# Autodesk Inventor assembly: Helix DLP
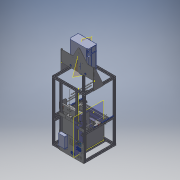
[picture p0: Inventor's stored thumbnail of the model, 180x180]
Saved by Autodesk Inventor 2019 (Build 230136000, 136)
## iProperties
Created: 2020-03-07
Part Number: Helix DLP
Document SubType Name: Assembly
Designer: Vijay
Author: Vijay
## Documents named in this file (32)
- C:\Users\Vijay\Documents\CAD Files\Helix DLP\Helix DLP.iam
- C:\Users\Vijay\Documents\CAD Files\Helix DLP\Helix DLP Z Stage.iam
- C:\Users\Vijay\Documents\CAD Files\Helix DLP\mgn12-linear-guide-subassembly-with-configurable-rail-length-1.snapshot.8\MGN12 LINEAR GUIDE RAIL, CONFIGURABLE, 500 mm.ipt
- C:\Users\Vijay\Documents\CAD Files\Helix DLP\3030-aluminum-extrusion-profile-2.snapshot.4\30X30 - T-slot - Aluminium Profile.ipt
- C:\Users\Vijay\Documents\CAD Files\Helix DLP\3030-aluminum-extrusion-profile-2.snapshot.4\30X30 - T-slot - Aluminium Profile_CPY.ipt
- C:\Users\Vijay\Documents\CAD Files\Helix DLP\3030-aluminum-extrusion-profile-2.snapshot.4\30X30 - T-slot - Aluminium Profile_CPY_CPY.ipt
- C:\Users\Vijay\Documents\CAD Files\Helix DLP\M1173041- NEMA 17 Screw rod.ipt
- C:\Users\Vijay\Documents\CAD Files\Helix DLP\Motor Brace_1.ipt
- C:\Users\Vijay\Documents\CAD Files\Helix DLP\Motor_brace_2.ipt
- C:\Users\Vijay\Documents\CAD Files\Helix DLP\motor_brace_3.ipt
- C:\Users\Vijay\Documents\CAD Files\Helix DLP\Tank2.ipt
- C:\Users\Vijay\Documents\CAD Files\Helix DLP\3030-aluminum-extrusion-profile-2.snapshot.4\30X30 - T-slot - Aluminium Profile_CPY_CPY_CPY.ipt
- C:\Users\Vijay\Documents\CAD Files\Helix DLP\mgn12-linear-guide-subassembly-with-configurable-rail-length-1.snapshot.8\MGN12H, LINEAR GUIDE BLOCK.ipt
- C:\Users\Vijay\Documents\CAD Files\Helix DLP\Wiper_Arm_1.ipt
- C:\Users\Vijay\Documents\CAD Files\Helix DLP\mgn12-linear-guide-subassembly-with-configurable-rail-length-1.snapshot.8\MGN12 LINEAR GUIDE RAIL, CONFIGURABLE, 500 mm_CPY.ipt
- C:\Users\Vijay\Documents\CAD Files\Helix DLP\wiper motor holder.ipt
- C:\Users\Vijay\Documents\CAD Files\Julia Extended Rev19\Julia Chassi(Chamfered)\Julia Chassi(Chamfered)\Julia 3D model\Z Motor Screw.ipt
- C:\Users\Vijay\Documents\CAD Files\Helix DLP\Wiper nut holder.ipt
- C:\Users\Vijay\Documents\CAD Files\Helix DLP\Rain T Slot.ipt
- C:\Users\Vijay\Documents\CAD Files\Helix DLP\Projector.ipt
- C:\Users\Vijay\Documents\CAD Files\Helix DLP\ProjectorMount 1.ipt
- C:\Users\Vijay\Documents\CAD Files\Helix DLP\Projector mount side.ipt
- C:\Users\Vijay\Documents\CAD Files\Helix DLP\SIde Actylic.ipt
- C:\Users\Vijay\Documents\CAD Files\Helix DLP\wiper.ipt
- C:\Users\Vijay\Documents\CAD Files\Helix DLP\wiper 2.ipt
- C:\Users\Vijay\Documents\CAD Files\Helix DLP\Electronics Base.ipt
- C:\Users\Vijay\Documents\CAD Files\Helix DLP\ArduinoUno.ipt
- C:\Users\Vijay\Documents\CAD Files\Helix DLP\V8_AC switch_1.ipt
- C:\Users\Vijay\Documents\CAD Files\Helix DLP\Raspberry Pi 3 Model B+ Reference Model.ipt
- C:\Users\Vijay\Documents\CAD Files\Helix DLP\24v Smps.ipt
- C:\Users\Vijay\Documents\CAD Files\Helix DLP\Limit Switch (1).ipt
- C:\Users\Vijay\Documents\CAD Files\Helix DLP\Z limit switch holder.ipt
## Components (60 placed, 31 different names)
1. Helix DLP Z Stage:1 [sub-assembly] — Mate:1, Mate:2, Mate:3, Mate:19, Angle:1, Mate:34, Mate:35, Angle:4
2. MGN12 LINEAR GUIDE RAIL, CONFIGURABLE, 500 mm:1 — Flush:1, Flush:2, Mate:3, Mate:4, Flush:13
3. MGN12 LINEAR GUIDE RAIL, CONFIGURABLE, 500 mm:2 — Flush:1, Flush:2, Mate:1, Mate:2, Mate:5, Flush:14, Flush:15
4. 30X30 - T-slot - Aluminium Profile:1 — Mate:5, Flush:7, Flush:9, Flush:14, Flush:15, Mate:7, Mate:87, Flush:81, Flush:82
5. 30X30 - T-slot - Aluminium Profile:2 — Mate:4, Flush:8, Flush:13, Mate:6, Flush:17, Flush:39
6. 30X30 - T-slot - Aluminium Profile:3 — Flush:4, Flush:5, Flush:7, Flush:9, Flush:11, Mate:7, Mate:8, Flush:18, Flush:19, Mate:10, Flush:36, Flush:56, Mate:50, Flush:80
7. 30X30 - T-slot - Aluminium Profile:4 — Flush:4, Flush:8, Flush:10, Mate:6, Flush:17, Mate:72
8. 30X30 - T-slot - Aluminium Profile:5 — Flush:5, Flush:6, Flush:10, Flush:12, Flush:20, Flush:21, Flush:25, Flush:37, Mate:17, Mate:22, Flush:44, Mate:43
9. 30X30 - T-slot - Aluminium Profile:6 — Flush:6, Flush:11, Flush:12, Mate:9, Mate:10, Mate:16, Flush:32, Flush:33, Mate:18, Mate:23, Flush:45, Mate:41, Flush:74
10. 30X30 - T-slot - Aluminium Profile_CPY:1 — Mate:8, Flush:18, Flush:19
11. 30X30 - T-slot - Aluminium Profile_CPY:2 — Flush:20, Flush:21, Mate:9, Mate:11, Flush:22, Flush:23, Flush:24, Mate:12
12. 30X30 - T-slot - Aluminium Profile_CPY_CPY:1 — Mate:11, Flush:22, Flush:23
13. 30X30 - T-slot - Aluminium Profile_CPY_CPY:2 — Flush:24, Mate:12, Flush:25, Flush:67
14. 30X30 - T-slot - Aluminium Profile_CPY:3 — Flush:30, Mate:15, Flush:31, Flush:79
15. 30X30 - T-slot - Aluminium Profile_CPY:4 — Flush:29, Mate:16, Flush:32, Mate:37, Flush:53
16. 30X30 - T-slot - Aluminium Profile_CPY_CPY:3 — Flush:31, Flush:33, Mate:38
17. 30X30 - T-slot - Aluminium Profile_CPY_CPY:4 — Flush:29, Flush:30, Mate:15, Mate:39
18. 30X30 - T-slot - Aluminium Profile_CPY_CPY:5 — Flush:37, Mate:17, Flush:38, Flush:55, Mate:42
19. 30X30 - T-slot - Aluminium Profile_CPY_CPY:6 — Flush:36, Mate:18, Flush:38, Mate:40, Flush:54, Mate:47
20. M1173041- NEMA 17 Screw rod:1 — Mate:19, Angle:1, Flush:40
21. Motor Brace_1:1 — Flush:39, Mate:21
22. Motor_brace_2:1 — Flush:40, Flush:41, Mate:20, Flush:42
23. motor_brace_3:1 — Flush:41
24. motor_brace_3:2 — Mate:20, Mate:21, Flush:42
25. Tank2:1 — Mate:24, Mate:33, Mate:34, Mate:35, Angle:3, Mate:68
26. 30X30 - T-slot - Aluminium Profile_CPY_CPY_CPY:1 — Mate:22, Flush:44, Flush:46, Flush:65
27. 30X30 - T-slot - Aluminium Profile_CPY_CPY_CPY:2 — Mate:23, Flush:45, Flush:46, Mate:24
28. MGN12H, LINEAR GUIDE BLOCK:1 — Flush:49, Mate:45, Mate:73
29. MGN12H, LINEAR GUIDE BLOCK:2 — Flush:49, Flush:50, Mate:44, Mate:48, Mate:64, Mate:65
30. Wiper_Arm_1:1 — Flush:50, Mate:33, Mate:51, Mate:52, Flush:59, Flush:61, Mate:64, Mate:65, Flush:77
31. 30X30 - T-slot - Aluminium Profile_CPY_CPY:7 — Flush:51, Mate:38
32. 30X30 - T-slot - Aluminium Profile_CPY_CPY:8 — Flush:51, Mate:37, Flush:53, Mate:39
33. M1173041- NEMA 17 Screw rod:2 — Mate:47, Mate:49, Mate:50, Flush:57, Flush:60, Mate:55
34. MGN12 LINEAR GUIDE RAIL, CONFIGURABLE, 500 mm_CPY:1 — Mate:40, Flush:54, Mate:41, Mate:44, Mate:48
35. MGN12 LINEAR GUIDE RAIL, CONFIGURABLE, 500 mm_CPY:2 — Flush:55, Mate:42, Mate:43, Mate:45, Mate:73
36. wiper motor holder:1 — Flush:56, Mate:49, Flush:57
37. Z Motor Screw:1 — Mate:53, Mate:54, Mate:55, Mate:56
38. motor_brace_3:3 — Mate:52, Flush:58, Flush:59
39. motor_brace_3:4 — Mate:51, Flush:58, Flush:60, Flush:61, Flush:62, Angle:2
40. Wiper nut holder:1 — Flush:62, Mate:53, Mate:54, Mate:56, Angle:2
41. Rain T Slot:1 — Flush:65
42. Projector:1 — Angle:3, Angle:4, Mate:68, Flush:68, Mate:70, Angle:5, Mate:74
43. ProjectorMount 1:1 — Flush:67, Flush:68, Flush:69, Mate:69, Flush:72, Flush:73, Mate:71, Mate:74
44. Projector mount side:1 — Flush:69, Flush:70, Flush:71
45. Projector mount side:2 — Flush:70, Flush:71, Mate:69, Flush:72, Flush:73
46. SIde Actylic:1 — Flush:74, Flush:75, Flush:76
47. SIde Actylic:2 — Mate:72, Flush:75, Flush:76
48. wiper:1 — Flush:77, Flush:78
49. wiper 2:1 — Flush:78
50. Rain T Slot:2
51. Rain T Slot:3
52. Rain T Slot:4
53. Electronics Base:1 — Mate:75, Mate:76, Mate:77, Mate:78, Mate:79, Mate:80, Mate:81, Mate:82, Mate:83, Mate:84, Mate:85, Mate:86, Mate:87, Flush:79, Flush:80
54. ArduinoUno:1 — Mate:76, Mate:77, Mate:85
55. V8_AC switch_1:1 — Mate:81, Mate:82, Mate:84
56. Raspberry Pi 3 Model B+ Reference Model:1 — Mate:78, Mate:79, Mate:86
57. 24v Smps:1 — Mate:75, Mate:80, Mate:83
58. Limit Switch (1):1
59. Limit Switch (1):2
60. Z limit switch holder:1 — Flush:81, Flush:82
## Relationships (144: Flush 71, Mate 68, Angle 5)
- Flush:1: MGN12 LINEAR GUIDE RAIL, CONFIGURABLE, 500 mm:1 ↔ MGN12 LINEAR GUIDE RAIL, CONFIGURABLE, 500 mm:2
- Flush:2: MGN12 LINEAR GUIDE RAIL, CONFIGURABLE, 500 mm:1 ↔ MGN12 LINEAR GUIDE RAIL, CONFIGURABLE, 500 mm:2
- Mate:1: Helix DLP Z Stage:1 ↔ MGN12 LINEAR GUIDE RAIL, CONFIGURABLE, 500 mm:2
- Mate:2: Helix DLP Z Stage:1 ↔ MGN12 LINEAR GUIDE RAIL, CONFIGURABLE, 500 mm:2
- Mate:3: Helix DLP Z Stage:1 ↔ MGN12 LINEAR GUIDE RAIL, CONFIGURABLE, 500 mm:1
- Mate:4: MGN12 LINEAR GUIDE RAIL, CONFIGURABLE, 500 mm:1 ↔ 30X30 - T-slot - Aluminium Profile:2
- Mate:5: MGN12 LINEAR GUIDE RAIL, CONFIGURABLE, 500 mm:2 ↔ 30X30 - T-slot - Aluminium Profile:1
- Flush:4: 30X30 - T-slot - Aluminium Profile:3 ↔ 30X30 - T-slot - Aluminium Profile:4
- Flush:5: 30X30 - T-slot - Aluminium Profile:3 ↔ 30X30 - T-slot - Aluminium Profile:5
- Flush:6: 30X30 - T-slot - Aluminium Profile:5 ↔ 30X30 - T-slot - Aluminium Profile:6
- Flush:7: 30X30 - T-slot - Aluminium Profile:1 ↔ 30X30 - T-slot - Aluminium Profile:3
- Flush:8: 30X30 - T-slot - Aluminium Profile:2 ↔ 30X30 - T-slot - Aluminium Profile:4
- Flush:9: 30X30 - T-slot - Aluminium Profile:1 ↔ 30X30 - T-slot - Aluminium Profile:3
- Flush:10: 30X30 - T-slot - Aluminium Profile:4 ↔ 30X30 - T-slot - Aluminium Profile:5
- Flush:11: 30X30 - T-slot - Aluminium Profile:3 ↔ 30X30 - T-slot - Aluminium Profile:6
- Flush:12: 30X30 - T-slot - Aluminium Profile:5 ↔ 30X30 - T-slot - Aluminium Profile:6
- Flush:13 (9.0175 mm): MGN12 LINEAR GUIDE RAIL, CONFIGURABLE, 500 mm:1 ↔ 30X30 - T-slot - Aluminium Profile:2
- Flush:14 (9.0175 mm): MGN12 LINEAR GUIDE RAIL, CONFIGURABLE, 500 mm:2 ↔ 30X30 - T-slot - Aluminium Profile:1
- Flush:15 (-50 mm): MGN12 LINEAR GUIDE RAIL, CONFIGURABLE, 500 mm:2 ↔ 30X30 - T-slot - Aluminium Profile:1
- Mate:6 (100 mm): 30X30 - T-slot - Aluminium Profile:2 ↔ 30X30 - T-slot - Aluminium Profile:4
- Mate:7 (100 mm): 30X30 - T-slot - Aluminium Profile:1 ↔ 30X30 - T-slot - Aluminium Profile:3
- Flush:17: 30X30 - T-slot - Aluminium Profile:2 ↔ 30X30 - T-slot - Aluminium Profile:4
- Mate:8: 30X30 - T-slot - Aluminium Profile:3 ↔ 30X30 - T-slot - Aluminium Profile_CPY:1
- Flush:18: 30X30 - T-slot - Aluminium Profile:3 ↔ 30X30 - T-slot - Aluminium Profile_CPY:1
- Flush:19: 30X30 - T-slot - Aluminium Profile:3 ↔ 30X30 - T-slot - Aluminium Profile_CPY:1
- Flush:20: 30X30 - T-slot - Aluminium Profile:5 ↔ 30X30 - T-slot - Aluminium Profile_CPY:2
- Flush:21: 30X30 - T-slot - Aluminium Profile:5 ↔ 30X30 - T-slot - Aluminium Profile_CPY:2
- Mate:9: 30X30 - T-slot - Aluminium Profile:6 ↔ 30X30 - T-slot - Aluminium Profile_CPY:2
- Mate:10 (500 mm): 30X30 - T-slot - Aluminium Profile:3 ↔ 30X30 - T-slot - Aluminium Profile:6
- Mate:11: 30X30 - T-slot - Aluminium Profile_CPY:2 ↔ 30X30 - T-slot - Aluminium Profile_CPY_CPY:1
- Flush:22: 30X30 - T-slot - Aluminium Profile_CPY:2 ↔ 30X30 - T-slot - Aluminium Profile_CPY_CPY:1
- Flush:23: 30X30 - T-slot - Aluminium Profile_CPY:2 ↔ 30X30 - T-slot - Aluminium Profile_CPY_CPY:1
- Flush:24: 30X30 - T-slot - Aluminium Profile_CPY:2 ↔ 30X30 - T-slot - Aluminium Profile_CPY_CPY:2
- Mate:12: 30X30 - T-slot - Aluminium Profile_CPY:2 ↔ 30X30 - T-slot - Aluminium Profile_CPY_CPY:2
- Flush:25: 30X30 - T-slot - Aluminium Profile:5 ↔ 30X30 - T-slot - Aluminium Profile_CPY_CPY:2
- [Mate]: 30X30 - T-slot - Aluminium Profile_CPY:4 ↔ 30X30 - T-slot - Aluminium Profile_CPY_CPY:3
- [Flush]: 30X30 - T-slot - Aluminium Profile_CPY:4 ↔ 30X30 - T-slot - Aluminium Profile_CPY_CPY:3
- [Flush]: 30X30 - T-slot - Aluminium Profile_CPY:4 ↔ 30X30 - T-slot - Aluminium Profile_CPY_CPY:3
- [Flush]: 30X30 - T-slot - Aluminium Profile_CPY:4 ↔ 30X30 - T-slot - Aluminium Profile_CPY_CPY:4
- [Mate]: 30X30 - T-slot - Aluminium Profile_CPY:4 ↔ 30X30 - T-slot - Aluminium Profile_CPY_CPY:4
- Flush:29: 30X30 - T-slot - Aluminium Profile_CPY:4 ↔ 30X30 - T-slot - Aluminium Profile_CPY_CPY:4
- Flush:30: 30X30 - T-slot - Aluminium Profile_CPY:3 ↔ 30X30 - T-slot - Aluminium Profile_CPY_CPY:4
- Mate:15: 30X30 - T-slot - Aluminium Profile_CPY:3 ↔ 30X30 - T-slot - Aluminium Profile_CPY_CPY:4
- Mate:16: 30X30 - T-slot - Aluminium Profile:6 ↔ 30X30 - T-slot - Aluminium Profile_CPY:4
- Flush:31: 30X30 - T-slot - Aluminium Profile_CPY:3 ↔ 30X30 - T-slot - Aluminium Profile_CPY_CPY:3
- Flush:32: 30X30 - T-slot - Aluminium Profile:6 ↔ 30X30 - T-slot - Aluminium Profile_CPY:4
- Flush:33: 30X30 - T-slot - Aluminium Profile:6 ↔ 30X30 - T-slot - Aluminium Profile_CPY_CPY:3
- Flush:36: 30X30 - T-slot - Aluminium Profile:3 ↔ 30X30 - T-slot - Aluminium Profile_CPY_CPY:6
- Flush:37: 30X30 - T-slot - Aluminium Profile:5 ↔ 30X30 - T-slot - Aluminium Profile_CPY_CPY:5
- Mate:17: 30X30 - T-slot - Aluminium Profile:5 ↔ 30X30 - T-slot - Aluminium Profile_CPY_CPY:5
- Mate:18: 30X30 - T-slot - Aluminium Profile:6 ↔ 30X30 - T-slot - Aluminium Profile_CPY_CPY:6
- Flush:38: 30X30 - T-slot - Aluminium Profile_CPY_CPY:5 ↔ 30X30 - T-slot - Aluminium Profile_CPY_CPY:6
- Mate:19: Helix DLP Z Stage:1 ↔ M1173041- NEMA 17 Screw rod:1
- Flush:39: 30X30 - T-slot - Aluminium Profile:2 ↔ Motor Brace_1:1
- Angle:1 (0 deg): Helix DLP Z Stage:1 ↔ M1173041- NEMA 17 Screw rod:1
- Flush:40: M1173041- NEMA 17 Screw rod:1 ↔ Motor_brace_2:1
- Flush:41: Motor_brace_2:1 ↔ motor_brace_3:1
- Mate:20: Motor_brace_2:1 ↔ motor_brace_3:2
- Mate:21: Motor Brace_1:1 ↔ motor_brace_3:2
- Flush:42: Motor_brace_2:1 ↔ motor_brace_3:2
- Mate:22: 30X30 - T-slot - Aluminium Profile:5 ↔ 30X30 - T-slot - Aluminium Profile_CPY_CPY_CPY:1
- Flush:44: 30X30 - T-slot - Aluminium Profile:5 ↔ 30X30 - T-slot - Aluminium Profile_CPY_CPY_CPY:1
- Mate:23: 30X30 - T-slot - Aluminium Profile:6 ↔ 30X30 - T-slot - Aluminium Profile_CPY_CPY_CPY:2
- Flush:45: 30X30 - T-slot - Aluminium Profile:6 ↔ 30X30 - T-slot - Aluminium Profile_CPY_CPY_CPY:2
- Flush:46: 30X30 - T-slot - Aluminium Profile_CPY_CPY_CPY:1 ↔ 30X30 - T-slot - Aluminium Profile_CPY_CPY_CPY:2
- Mate:24: Tank2:1 ↔ 30X30 - T-slot - Aluminium Profile_CPY_CPY_CPY:2
- Flush:49: MGN12H, LINEAR GUIDE BLOCK:1 ↔ MGN12H, LINEAR GUIDE BLOCK:2
- Flush:50: MGN12H, LINEAR GUIDE BLOCK:2 ↔ Wiper_Arm_1:1
- Mate:33 (9 mm): Tank2:1 ↔ Wiper_Arm_1:1
- Mate:34 (10 mm): Helix DLP Z Stage:1 ↔ Tank2:1
- Mate:35 (10 mm): Helix DLP Z Stage:1 ↔ Tank2:1
- Flush:51: 30X30 - T-slot - Aluminium Profile_CPY_CPY:7 ↔ 30X30 - T-slot - Aluminium Profile_CPY_CPY:8
- Mate:37: 30X30 - T-slot - Aluminium Profile_CPY:4 ↔ 30X30 - T-slot - Aluminium Profile_CPY_CPY:8
- Flush:53: 30X30 - T-slot - Aluminium Profile_CPY:4 ↔ 30X30 - T-slot - Aluminium Profile_CPY_CPY:8
- Mate:38 (120 mm): 30X30 - T-slot - Aluminium Profile_CPY_CPY:3 ↔ 30X30 - T-slot - Aluminium Profile_CPY_CPY:7
- Mate:39 (120 mm): 30X30 - T-slot - Aluminium Profile_CPY_CPY:4 ↔ 30X30 - T-slot - Aluminium Profile_CPY_CPY:8
- Mate:40: 30X30 - T-slot - Aluminium Profile_CPY_CPY:6 ↔ MGN12 LINEAR GUIDE RAIL, CONFIGURABLE, 500 mm_CPY:1
- Flush:54 (9.018 mm): 30X30 - T-slot - Aluminium Profile_CPY_CPY:6 ↔ MGN12 LINEAR GUIDE RAIL, CONFIGURABLE, 500 mm_CPY:1
- Mate:41: 30X30 - T-slot - Aluminium Profile:6 ↔ MGN12 LINEAR GUIDE RAIL, CONFIGURABLE, 500 mm_CPY:1
- Flush:55 (9.018 mm): 30X30 - T-slot - Aluminium Profile_CPY_CPY:5 ↔ MGN12 LINEAR GUIDE RAIL, CONFIGURABLE, 500 mm_CPY:2
- Mate:42: 30X30 - T-slot - Aluminium Profile_CPY_CPY:5 ↔ MGN12 LINEAR GUIDE RAIL, CONFIGURABLE, 500 mm_CPY:2
- Mate:43: 30X30 - T-slot - Aluminium Profile:5 ↔ MGN12 LINEAR GUIDE RAIL, CONFIGURABLE, 500 mm_CPY:2
- Mate:44: MGN12H, LINEAR GUIDE BLOCK:2 ↔ MGN12 LINEAR GUIDE RAIL, CONFIGURABLE, 500 mm_CPY:1
- Mate:45: MGN12H, LINEAR GUIDE BLOCK:1 ↔ MGN12 LINEAR GUIDE RAIL, CONFIGURABLE, 500 mm_CPY:2
- Flush:56: 30X30 - T-slot - Aluminium Profile:3 ↔ wiper motor holder:1
- Mate:47 (20 mm): 30X30 - T-slot - Aluminium Profile_CPY_CPY:6 ↔ M1173041- NEMA 17 Screw rod:2
- Mate:48: MGN12H, LINEAR GUIDE BLOCK:2 ↔ MGN12 LINEAR GUIDE RAIL, CONFIGURABLE, 500 mm_CPY:1
- Mate:49: M1173041- NEMA 17 Screw rod:2 ↔ wiper motor holder:1
- Mate:50 (5 mm): 30X30 - T-slot - Aluminium Profile:3 ↔ M1173041- NEMA 17 Screw rod:2
- Flush:57 (4 mm): M1173041- NEMA 17 Screw rod:2 ↔ wiper motor holder:1
- Mate:51: Wiper_Arm_1:1 ↔ motor_brace_3:4
- Mate:52: Wiper_Arm_1:1 ↔ motor_brace_3:3
- Flush:58: motor_brace_3:3 ↔ motor_brace_3:4
- Flush:59: Wiper_Arm_1:1 ↔ motor_brace_3:3
- Flush:60 (-0.106 mm): M1173041- NEMA 17 Screw rod:2 ↔ motor_brace_3:4
- Flush:61 (4 mm): Wiper_Arm_1:1 ↔ motor_brace_3:4
- Flush:62: motor_brace_3:4 ↔ Wiper nut holder:1
- Mate:53: Z Motor Screw:1 ↔ Wiper nut holder:1
- Mate:54: Z Motor Screw:1 ↔ Wiper nut holder:1
- Mate:55: M1173041- NEMA 17 Screw rod:2 ↔ Z Motor Screw:1
- Mate:56: Z Motor Screw:1 ↔ Wiper nut holder:1
- Flush:65: 30X30 - T-slot - Aluminium Profile_CPY_CPY_CPY:1 ↔ Rain T Slot:1
- Mate:64: MGN12H, LINEAR GUIDE BLOCK:2 ↔ Wiper_Arm_1:1
- Mate:65: MGN12H, LINEAR GUIDE BLOCK:2 ↔ Wiper_Arm_1:1
- Angle:2 (0 deg): motor_brace_3:4 ↔ Wiper nut holder:1
- Angle:3 (180 deg): Tank2:1 ↔ Projector:1
- Angle:4 (180 deg): Helix DLP Z Stage:1 ↔ Projector:1
- Mate:68 (750 mm): Tank2:1 ↔ Projector:1
- Flush:67: 30X30 - T-slot - Aluminium Profile_CPY_CPY:2 ↔ ProjectorMount 1:1
- Flush:68: Projector:1 ↔ ProjectorMount 1:1
- Flush:69: ProjectorMount 1:1 ↔ Projector mount side:1
- Flush:70: Projector mount side:1 ↔ Projector mount side:2
- Flush:71: Projector mount side:1 ↔ Projector mount side:2
- Mate:69: ProjectorMount 1:1 ↔ Projector mount side:2
- Flush:72 (10 mm): ProjectorMount 1:1 ↔ Projector mount side:2
- Flush:73 (-10 mm): ProjectorMount 1:1 ↔ Projector mount side:2
- Mate:70: Projector:1
- Angle:5 (0 deg): Projector:1
- Mate:71: ProjectorMount 1:1
- Flush:74: 30X30 - T-slot - Aluminium Profile:6 ↔ SIde Actylic:1
- Mate:72: 30X30 - T-slot - Aluminium Profile:4 ↔ SIde Actylic:2
- Flush:75: SIde Actylic:1 ↔ SIde Actylic:2
- Flush:76: SIde Actylic:1 ↔ SIde Actylic:2
- Mate:73: MGN12H, LINEAR GUIDE BLOCK:1 ↔ MGN12 LINEAR GUIDE RAIL, CONFIGURABLE, 500 mm_CPY:2
- Mate:74: Projector:1 ↔ ProjectorMount 1:1
- Flush:77: Wiper_Arm_1:1 ↔ wiper:1
- Flush:78: wiper:1 ↔ wiper 2:1
- Mate:75: Electronics Base:1 ↔ 24v Smps:1
- Mate:76: Electronics Base:1 ↔ ArduinoUno:1
- Mate:77: Electronics Base:1 ↔ ArduinoUno:1
- Mate:78: Electronics Base:1 ↔ Raspberry Pi 3 Model B+ Reference Model:1
- Mate:79: Electronics Base:1 ↔ Raspberry Pi 3 Model B+ Reference Model:1
- Mate:80: Electronics Base:1 ↔ 24v Smps:1
- Mate:81: Electronics Base:1 ↔ V8_AC switch_1:1
- Mate:82: Electronics Base:1 ↔ V8_AC switch_1:1
- Mate:83: Electronics Base:1 ↔ 24v Smps:1
- Mate:84: Electronics Base:1 ↔ V8_AC switch_1:1
- Mate:85: Electronics Base:1 ↔ ArduinoUno:1
- Mate:86: Electronics Base:1 ↔ Raspberry Pi 3 Model B+ Reference Model:1
- Mate:87: 30X30 - T-slot - Aluminium Profile:1 ↔ Electronics Base:1
- Flush:79: 30X30 - T-slot - Aluminium Profile_CPY:3 ↔ Electronics Base:1
- Flush:80: 30X30 - T-slot - Aluminium Profile:3 ↔ Electronics Base:1
- Flush:81: 30X30 - T-slot - Aluminium Profile:1 ↔ Z limit switch holder:1
- Flush:82: 30X30 - T-slot - Aluminium Profile:1 ↔ Z limit switch holder:1
## Named parameters: d41_d35 = 0 mm, d42_d36 = 0 mm, d43_d37 = 0 mm, d44_d38 = 0 mm, d45_d39 = 0 mm
